# Autodesk Inventor assembly: PotentiometerPlacement
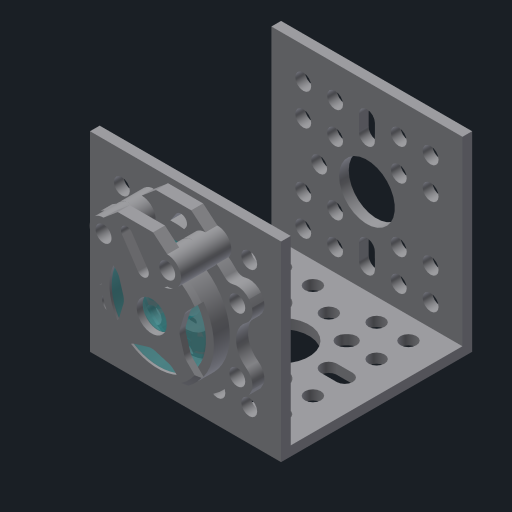
[picture p0: Inventor's stored thumbnail of the model, 512x512]
Saved by Autodesk Inventor 2023 (Build 270158000, 158)
## iProperties
Created: 2023-09-23
Part Number: PotentiometerPlacement
Document SubType Name: Assembly
Designer: valer
Author: valer
## Documents named in this file (5)
- C:\Users\valer\Desktop\str1ker\cad\PotentiometerPlacement.iam
- C:\Users\valer\Desktop\str1ker\cad\external\ShoulderBracket.ipt
- C:\Users\valer\Desktop\str1ker\cad\PotentiometerCover.ipt
- C:\Users\valer\Desktop\str1ker\cad\external\Potentiometer\Body.ipt
- C:\Users\valer\Desktop\str1ker\cad\PotentiometerBracketBase.ipt
## Components (5 placed, 4 different names)
1. ShoulderServoBracket:1 — Mate:2, Mate:3, Mate:4, Mate:5, Angle:1, Mate:7, Mate:8, Mate:13
2. PotentiometerCover:1 — Mate:2, Mate:3, Mate:4, Mate:6
3. Body:1 — Mate:5, Mate:6, Angle:1
4. PotentiometerBracketBase:1 — Mate:7, Mate:8, Mate:13, Mate:15, Mate:16, Mate:17
5. PotentiometerBracketBase:2 — Mate:15, Mate:16, Mate:17
## Relationships (12: Mate 11, Angle 1)
- Mate:2: ShoulderServoBracket:1 ↔ PotentiometerCover:1
- Mate:3: ShoulderServoBracket:1 ↔ PotentiometerCover:1
- Mate:4: ShoulderServoBracket:1 ↔ PotentiometerCover:1
- Mate:5: ShoulderServoBracket:1 ↔ Body:1
- Mate:6: PotentiometerCover:1 ↔ Body:1
- Angle:1 (0 deg): ShoulderServoBracket:1 ↔ Body:1
- Mate:7: ShoulderServoBracket:1 ↔ PotentiometerBracketBase:1
- Mate:8: ShoulderServoBracket:1 ↔ PotentiometerBracketBase:1
- Mate:13: ShoulderServoBracket:1 ↔ PotentiometerBracketBase:1
- Mate:15: PotentiometerBracketBase:1 ↔ PotentiometerBracketBase:2
- Mate:16: PotentiometerBracketBase:1 ↔ PotentiometerBracketBase:2
- Mate:17: PotentiometerBracketBase:1 ↔ PotentiometerBracketBase:2
